# Autodesk Inventor assembly: sch40conduit
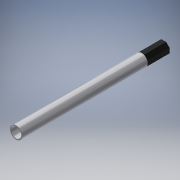
[picture p0: Inventor's stored thumbnail of the model, 180x180]
Saved by Autodesk Inventor 2017 (Build 210142000, 142)
## iProperties
Created: 2018-11-30
Part Number: sch40conduit
Document SubType Name: Assembly
Designer: ddeboer
Author: ddeboer
## Documents named in this file (3)
- C:\Users\ddeboer\Desktop\sch40_conduit\sch40conduit.iam
- C:\Users\ddeboer\Desktop\sch40_conduit\conduit_endcap.ipt
- C:\Users\ddeboer\Desktop\sch40_conduit\outer_sheath.ipt
## Components (2 placed, 2 different names)
1. conduit_endcap:1 — Insert:1
2. outer_sheath:1 — Insert:1
## Relationships (1: Insert 1)
- Insert:1 (-25 mm): conduit_endcap:1 ↔ outer_sheath:1
